# Autodesk Inventor assembly: Podstawa+silnik
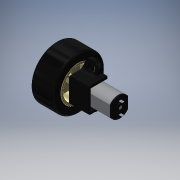
[picture p0: Inventor's stored thumbnail of the model, 180x180]
Saved by Autodesk Inventor 2017 (Build 210142000, 142)
## iProperties
Created: 2016-11-09
Part Number: Podstawa+silnik
Document SubType Name: Assembly
Designer: Shichi
Author: Shichi
## Documents named in this file (3)
- C:\Users\Shichi\Desktop\TooStronk\Podstawa+silnik.iam
- C:\Users\Shichi\Desktop\TooStronk\Koła\POLOLU+mocowanie.iam
- C:\Users\Shichi\Desktop\TooStronk\Koła\Kolo+Opona.iam
## Components (2 placed, 2 different names)
1. Kolo+Opona:2 [sub-assembly] — Insert:13
2. POLOLU+mocowanie:2 [sub-assembly] — Insert:13
## Relationships (1: Insert 1)
- Insert:13: Kolo+Opona:2 ↔ POLOLU+mocowanie:2
